# Autodesk Inventor assembly: Stepper Motor NEMA 17
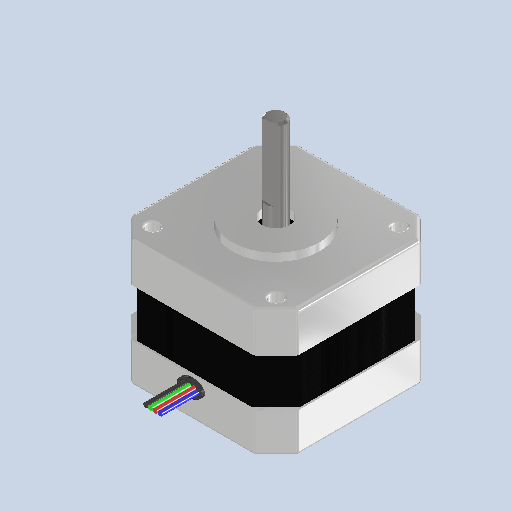
[picture p0: Inventor's stored thumbnail of the model, 512x512]
Saved by Autodesk Inventor 2025.1 (Build 291241000, 241)
## iProperties
Created: 2021-06-25
Part Number: Stepper Motor NEMA 17
Document SubType Name: Assembly
Designer: Work
Author: Work
## Documents named in this file (4)
- C:\Users\vedan\OneDrive\Desktop\Engineer 1P13\Design Studio\Project 1\files\Rotary Actuator Assembly\4. Rotary Actuator\Stepper Motor NEMA 17.iam
- C:\Users\vedan\OneDrive\Desktop\Engineer 1P13\Design Studio\Project 1\files\Rotary Actuator Assembly\4. Rotary Actuator\Piece1.ipt
- C:\Users\vedan\OneDrive\Desktop\Engineer 1P13\Design Studio\Project 1\files\Rotary Actuator Assembly\4. Rotary Actuator\Piece2.ipt
- C:\Users\vedan\OneDrive\Desktop\Engineer 1P13\Design Studio\Project 1\files\Rotary Actuator Assembly\4. Rotary Actuator\Stepper Motor Shaft.ipt
## Components (3 placed, 3 different names)
1. Piece1:1 — Mate:1, Flush:1, Flush:2, Insert:1, Flush:4
2. Piece2:1 — Mate:1, Flush:1, Flush:2
3. Stepper Motor Shaft:1 — Insert:1, Flush:3
## Relationships (6: Flush 4, Mate 1, Insert 1)
- Mate:1: Piece1:1 ↔ Piece2:1
- Flush:1: Piece1:1 ↔ Piece2:1
- Flush:2: Piece1:1 ↔ Piece2:1
- Insert:1: Piece1:1 ↔ Stepper Motor Shaft:1
- Flush:3: Stepper Motor Shaft:1
- Flush:4: Piece1:1
